# Autodesk Inventor assembly: BaseAssembly
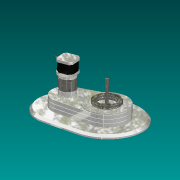
[picture p0: Inventor's stored thumbnail of the model, 180x180]
Saved by Autodesk Inventor 2020.2 (Build 242310000, 310)
## iProperties
Created: 2020-05-14
Part Number: BaseAssembly
Document SubType Name: Assembly
Designer: Svend
Author: Svend
## Documents named in this file (14)
- C:\Users\Svend\OneDrive\Documents\GitHub\BeerMinder\3D-model\Base (Axis 1)\BaseAssembly.iam
- C:\Users\Svend\OneDrive\Documents\GitHub\BeerMinder\3D-model\subAssembly\Nema17MetGearbox.iam
- C:\Users\Svend\OneDrive\Documents\GitHub\BeerMinder\3D-model\pulleys\GT2 Timing Pulley 20T - 8mm as.ipt
- C:\Users\Svend\OneDrive\Documents\GitHub\BeerMinder\3D-model\pulleys\GT2 Timing Pulley 60T - 8mm as.ipt
- C:\Users\Svend\OneDrive\Documents\Inventor\Content Center Files\R2020\en-US\ISO 4026\ISO 4026 - M4 x 8 - ISO.ipt
- C:\Users\Svend\OneDrive\Documents\GitHub\BeerMinder\3D-model\pulleys\Tandriem20naar60T.ipt
- C:\Users\Svend\OneDrive\Documents\GitHub\BeerMinder\3D-model\Base (Axis 1)\AsBase.ipt
- C:\Users\Svend\OneDrive\Documents\GitHub\BeerMinder\3D-model\bearings\Ball Bearing 608ZZ.ipt
- C:\Users\Svend\OneDrive\Documents\GitHub\BeerMinder\3D-model\Base (Axis 1)\motorplaat.ipt
- C:\Users\Svend\OneDrive\Documents\GitHub\BeerMinder\3D-model\gearbox\afstandsplaatje.ipt
- C:\Users\Svend\OneDrive\Documents\GitHub\BeerMinder\3D-model\Base (Axis 1)\spacerBase.ipt
- C:\Users\Svend\OneDrive\Documents\GitHub\BeerMinder\3D-model\Base (Axis 1)\onderkantBase.ipt
- C:\Users\Svend\OneDrive\Documents\GitHub\BeerMinder\3D-model\bearings\51110 Groefkogellager - 70 mm.iam
- C:\Users\Svend\OneDrive\Documents\GitHub\BeerMinder\3D-model\Base (Axis 1)\AxiaalLagerBevestiging.ipt
## Components (16 placed, 13 different names)
1. Nema17MetGearbox:1 [sub-assembly] — Mate:1, Mate:14, Mate:15, Mate:16, Mate:21, Angle:1
2. GT2 Timing Pulley 20T - 8mm as:1 — Mate:1, Mate:7, Mate:20
3. GT2 Timing Pulley 60T - 8mm as:1 — Mate:2, Mate:3, Mate:4, Mate:5, Mate:9, Mate:18, Mate:19, Mate:21, Mate:35
4. ISO 4026 M4 x 8:1 — Mate:3, Mate:5
5. ISO 4026 M4 x 8:2 — Mate:2, Mate:4
6. Tandriem20naar60T:1 — Mate:7, Mate:18, Mate:19, Mate:20
7. AsBase:1 — Mate:9, Mate:10, Mate:12, Flush:4, Mate:36, Mate:38
8. Ball Bearing 608ZZ:1 — Mate:10, Flush:2
9. motorplaat:1 — Mate:12, Mate:17, Flush:2, Mate:22, Mate:23, Mate:24, Angle:1, Mate:37, Mate:39, Mate:40
10. afstandsplaatje:1 — Mate:14, Mate:15, Mate:16, Mate:17
11. spacerBase:1 — Mate:22, Mate:23, Mate:24, Mate:25, Mate:26, Mate:27, Mate:31
12. spacerBase:2 — Mate:25, Mate:26, Mate:27, Mate:30, Mate:34
13. onderkantBase:1 — Mate:29, Mate:30, Mate:31, Flush:3, Mate:34
14. Ball Bearing 608ZZ:2 — Mate:29, Flush:3, Flush:4, Mate:35
15. 51110 Groefkogellager - 70 mm:1 [sub-assembly] — Mate:36, Mate:37
16. AxiaalLagerBevestiging:1 — Mate:38, Mate:39, Mate:40
## Relationships (37: Mate 33, Flush 3, Angle 1)
- Mate:1: Nema17MetGearbox:1 ↔ GT2 Timing Pulley 20T - 8mm as:1
- Mate:2: GT2 Timing Pulley 60T - 8mm as:1 ↔ ISO 4026 M4 x 8:2
- Mate:3: GT2 Timing Pulley 60T - 8mm as:1 ↔ ISO 4026 M4 x 8:1
- Mate:4 (-12.5 mm): GT2 Timing Pulley 60T - 8mm as:1 ↔ ISO 4026 M4 x 8:2
- Mate:5 (-12.5 mm): GT2 Timing Pulley 60T - 8mm as:1 ↔ ISO 4026 M4 x 8:1
- Mate:7: GT2 Timing Pulley 20T - 8mm as:1 ↔ Tandriem20naar60T:1
- Mate:9: GT2 Timing Pulley 60T - 8mm as:1 ↔ AsBase:1
- Mate:10: AsBase:1 ↔ Ball Bearing 608ZZ:1
- Mate:12: AsBase:1 ↔ motorplaat:1
- Mate:14: Nema17MetGearbox:1 ↔ afstandsplaatje:1
- Mate:15: Nema17MetGearbox:1 ↔ afstandsplaatje:1
- Mate:16: Nema17MetGearbox:1 ↔ afstandsplaatje:1
- Mate:17: motorplaat:1 ↔ afstandsplaatje:1
- Mate:18 (0.5 mm): GT2 Timing Pulley 60T - 8mm as:1 ↔ Tandriem20naar60T:1
- Mate:19: GT2 Timing Pulley 60T - 8mm as:1 ↔ Tandriem20naar60T:1
- Mate:20 (0.5 mm): GT2 Timing Pulley 20T - 8mm as:1 ↔ Tandriem20naar60T:1
- Mate:21: Nema17MetGearbox:1 ↔ GT2 Timing Pulley 60T - 8mm as:1
- Flush:2: Ball Bearing 608ZZ:1 ↔ motorplaat:1
- Mate:22: motorplaat:1 ↔ spacerBase:1
- Mate:23: motorplaat:1 ↔ spacerBase:1
- Mate:24: motorplaat:1 ↔ spacerBase:1
- Mate:25: spacerBase:1 ↔ spacerBase:2
- Mate:26: spacerBase:1 ↔ spacerBase:2
- Mate:27: spacerBase:1 ↔ spacerBase:2
- Mate:29: onderkantBase:1 ↔ Ball Bearing 608ZZ:2
- Mate:30: spacerBase:2 ↔ onderkantBase:1
- Mate:31: spacerBase:1 ↔ onderkantBase:1
- Flush:3: onderkantBase:1 ↔ Ball Bearing 608ZZ:2
- Flush:4: AsBase:1 ↔ Ball Bearing 608ZZ:2
- Mate:34: spacerBase:2 ↔ onderkantBase:1
- Mate:35: GT2 Timing Pulley 60T - 8mm as:1 ↔ Ball Bearing 608ZZ:2
- Angle:1 (180 deg): Nema17MetGearbox:1 ↔ motorplaat:1
- Mate:36: AsBase:1 ↔ 51110 Groefkogellager - 70 mm:1
- Mate:37: motorplaat:1 ↔ 51110 Groefkogellager - 70 mm:1
- Mate:38: AsBase:1 ↔ AxiaalLagerBevestiging:1
- Mate:39: motorplaat:1 ↔ AxiaalLagerBevestiging:1
- Mate:40: motorplaat:1 ↔ AxiaalLagerBevestiging:1
